# Autodesk Inventor assembly: yaw_motor_mount
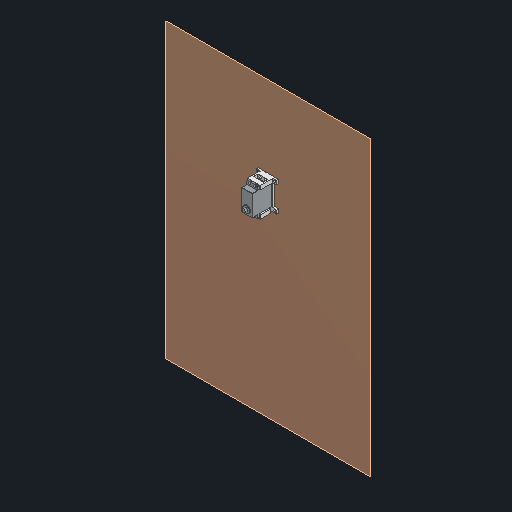
[picture p0: Inventor's stored thumbnail of the model, 512x512]
Saved by Autodesk Inventor 2026.1 (Build 301233020, 233B)
## iProperties
Created: 2025-11-24
Part Number: yaw_motor_mount
Document SubType Name: Assembly
Designer: jaewook
Author: jaewook
## Documents named in this file (3)
- C:\Users\kjh19\Documents\Inventor\project\proto2\example\yaw_motor_mount.iam
- C:\Users\kjh19\Documents\Inventor\project\proto2\example\yaw_motor_mount.ipt
- C:\Users\kjh19\Downloads\Servo+9imod+DS35MG-180\Servo-9imod-DS35MG-180.ipt
## Components (2 placed, 2 different names)
1. yaw_motor_mount:1 — 메이트:1
2. Servo-9imod-DS35MG-180:1 — 메이트:1
## Relationships (1: Mate 1)
- 메이트:1 [Mate]: yaw_motor_mount:1 ↔ Servo-9imod-DS35MG-180:1
